# Autodesk Inventor assembly: main_assy
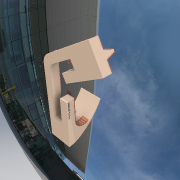
[picture p0: Inventor's stored thumbnail of the model, 180x180]
Saved by Autodesk Inventor 2019 (Build 230136000, 136)
## iProperties
Created: 2019-02-23
Part Number: main_assy
Document SubType Name: Assembly
Designer: gaincarlo
Author: gaincarlo
## Documents named in this file (14)
- D:\Giancarlo Bacchio\Documenti\00 - Progetti\30-Inventor\LaPanca-Baraca\main_assy.iam
- D:\Giancarlo Bacchio\Documenti\00 - Progetti\30-Inventor\LaPanca-Baraca\concrete_main.ipt
- D:\Giancarlo Bacchio\Documenti\00 - Progetti\30-Inventor\LaPanca-Baraca\solar_panel.ipt
- D:\Giancarlo Bacchio\Documenti\00 - Progetti\30-Inventor\LaPanca-Baraca\solar_panel_MIR.ipt
- D:\Giancarlo Bacchio\Documenti\00 - Progetti\30-Inventor\LaPanca-Baraca\curved-+_plates.iam
- D:\Giancarlo Bacchio\Documenti\00 - Progetti\30-Inventor\LaPanca-Baraca\curved-+_plates_MIR.iam
- D:\Giancarlo Bacchio\Documenti\00 - Progetti\30-Inventor\LaPanca-Baraca\back_plates.iam
- D:\Giancarlo Bacchio\Documenti\00 - Progetti\30-Inventor\LaPanca-Baraca\table_beam.ipt
- D:\Giancarlo Bacchio\Documenti\00 - Progetti\30-Inventor\LaPanca-Baraca\table_beam_MIR2.ipt
- D:\Giancarlo Bacchio\Documenti\00 - Progetti\30-Inventor\LaPanca-Baraca\table.iam
- D:\Giancarlo Bacchio\Documenti\00 - Progetti\30-Inventor\LaPanca-Baraca\angular30.ipt
- D:\Giancarlo Bacchio\Documenti\00 - Progetti\30-Inventor\LaPanca-Baraca\side_short.ipt
- D:\Giancarlo Bacchio\Documenti\00 - Progetti\30-Inventor\LaPanca-Baraca\table_inter.iam
- D:\Giancarlo Bacchio\Documenti\00 - Progetti\30-Inventor\LaPanca-Baraca\baraca.ipt
## Components (24 placed, 13 different names)
1. concrete_main:1 — Flush:4, Mate:1, Flush:5, Mate:2, Flush:6, Flush:7, Flush:8, Mate:3, Mate:4, Mate:5, Mate:6, Mate:7, Mate:8, Mate:12, Tangent:2, Flush:10
2. solar_panel:1
3. solar_panel_MIR:1
4. curved-+_plates:1 [sub-assembly] — Flush:4
5. curved-+_plates_MIR:1 [sub-assembly]
6. back_plates:2 [sub-assembly] — Flush:6, Flush:7, Flush:8
7. table_beam:1 — Mate:3, Mate:4, Mate:5
8. table_beam_MIR2:1 — Mate:6, Mate:7, Mate:8, Mate:9, Mate:10, Angle:1
9. table:1 [sub-assembly] — Mate:9, Mate:10, Angle:1
10. angular30:1 — Mate:11, Flush:9, Tangent:1, Mate:12, Tangent:2, Flush:10
11. angular30:2 — Mate:11, Flush:9, Tangent:1, Mate:13, Flush:11, Tangent:3
12. side_short:1 — Mate:13, Flush:11, Tangent:3, Flush:12, Flush:13, Mate:14, Flush:14, Flush:15, Mate:15, Flush:16, Mate:16, Mate:17, Flush:17, Mate:18, Mate:19, Mate:20, Mate:21, Mate:22, Mate:23, Mate:24, Mate:25, Flush:18, Flush:19, Mate:27
13. back_plates:4 [sub-assembly] — Flush:12, Flush:13, Mate:14
14. back_plates:7 [sub-assembly] — Flush:16, Mate:16, Mate:17
15. back_plates:8 [sub-assembly] — Flush:17, Mate:18, Mate:19
16. table_beam:2 — Mate:20, Mate:21, Mate:22, Mate:26, Angle:2
17. table_beam_MIR2:2 — Mate:23, Mate:24, Mate:25
18. table:2 [sub-assembly] — Mate:26, Angle:2
19. table_inter:1 [sub-assembly] — Flush:18, Flush:19, Mate:27
20. baraca:1
21. back_plates:1 [sub-assembly] — Mate:1, Flush:5, Mate:2
22. back_plates:3 [sub-assembly]
23. back_plates:5 [sub-assembly] — Flush:14, Flush:15, Mate:15
24. back_plates:6 [sub-assembly]
## Component patterns: (2 elements, first: back_plates:1), (2 elements, first: back_plates:5)
## Relationships (48: Mate 27, Flush 16, Tangent 3, Angle 2)
- Flush:4 (10 mm): concrete_main:1 ↔ curved-+_plates:1
- Mate:1 (10 mm): concrete_main:1 ↔ back_plates:1
- Flush:5: concrete_main:1 ↔ back_plates:1
- Mate:2 (-20 mm): concrete_main:1 ↔ back_plates:1
- Flush:6: concrete_main:1 ↔ back_plates:2
- Flush:7 (-20 mm): concrete_main:1 ↔ back_plates:2
- Flush:8 (-10 mm): concrete_main:1 ↔ back_plates:2
- Mate:3: concrete_main:1 ↔ table_beam:1
- Mate:4: concrete_main:1 ↔ table_beam:1
- Mate:5 (-250 mm): concrete_main:1 ↔ table_beam:1
- Mate:6: concrete_main:1 ↔ table_beam_MIR2:1
- Mate:7 (-250 mm): concrete_main:1 ↔ table_beam_MIR2:1
- Mate:8: concrete_main:1 ↔ table_beam_MIR2:1
- Mate:9: table_beam_MIR2:1 ↔ table:1
- Mate:10: table_beam_MIR2:1 ↔ table:1
- Angle:1 (0 deg): table_beam_MIR2:1 ↔ table:1
- Mate:11: angular30:1 ↔ angular30:2
- Flush:9: angular30:1 ↔ angular30:2
- Tangent:1: angular30:1 ↔ angular30:2
- Mate:12: concrete_main:1 ↔ angular30:1
- Tangent:2: concrete_main:1 ↔ angular30:1
- Flush:10: concrete_main:1 ↔ angular30:1
- Mate:13: angular30:2 ↔ side_short:1
- Flush:11: angular30:2 ↔ side_short:1
- Tangent:3: angular30:2 ↔ side_short:1
- Flush:12: side_short:1 ↔ back_plates:4
- Flush:13: side_short:1 ↔ back_plates:4
- Mate:14: side_short:1 ↔ back_plates:4
- Flush:14: side_short:1 ↔ back_plates:5
- Flush:15: side_short:1 ↔ back_plates:5
- Mate:15: side_short:1 ↔ back_plates:5
- Flush:16: side_short:1 ↔ back_plates:7
- Mate:16: side_short:1 ↔ back_plates:7
- Mate:17: side_short:1 ↔ back_plates:7
- Flush:17: side_short:1 ↔ back_plates:8
- Mate:18: side_short:1 ↔ back_plates:8
- Mate:19: side_short:1 ↔ back_plates:8
- Mate:20: side_short:1 ↔ table_beam:2
- Mate:21: side_short:1 ↔ table_beam:2
- Mate:22 (-250 mm): side_short:1 ↔ table_beam:2
- Mate:23: side_short:1 ↔ table_beam_MIR2:2
- Mate:24: side_short:1 ↔ table_beam_MIR2:2
- Mate:25 (-250 mm): side_short:1 ↔ table_beam_MIR2:2
- Mate:26: table_beam:2 ↔ table:2
- Angle:2 (0 deg): table_beam:2 ↔ table:2
- Flush:18: side_short:1 ↔ table_inter:1
- Flush:19: side_short:1 ↔ table_inter:1
- Mate:27: side_short:1 ↔ table_inter:1
